# Autodesk Inventor assembly: AssemblyGefreesdBasev2
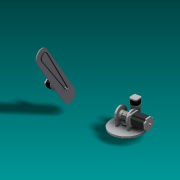
[picture p0: Inventor's stored thumbnail of the model, 180x180]
Saved by Autodesk Inventor 2020.2 (Build 242310000, 310)
## iProperties
Created: 2020-05-18
Part Number: AssemblyGefreesdBasev2
Document SubType Name: Assembly
Designer: Svend
Author: Svend
## Documents named in this file (20)
- C:\Users\Svend\OneDrive\Documents\GitHub\BeerMinder\3D-model\Base (Axis 1)\gefreesd\AssemblyGefreesdBasev2.iam
- C:\Users\Svend\OneDrive\Documents\GitHub\BeerMinder\3D-model\subAssembly\Nema17MetGearbox.iam
- C:\Users\Svend\OneDrive\Documents\GitHub\BeerMinder\3D-model\gearbox\afstandsplaatje.ipt
- C:\Users\Svend\OneDrive\Documents\GitHub\BeerMinder\3D-model\bearings\Ball Bearing 608ZZ.ipt
- C:\Users\Svend\OneDrive\Documents\GitHub\BeerMinder\3D-model\pulleys\GT2 Timing Pulley 20T - 8mm as.ipt
- C:\Users\Svend\OneDrive\Documents\GitHub\BeerMinder\3D-model\pulleys\GT2 Timing Pulley 60T - 8mm as.ipt
- C:\Users\Svend\OneDrive\Documents\GitHub\BeerMinder\3D-model\pulleys\Tandriem20naar60T.ipt
- C:\Users\Svend\OneDrive\Documents\GitHub\BeerMinder\3D-model\Base (Axis 1)\AsBase.ipt
- C:\Users\Svend\OneDrive\Documents\GitHub\BeerMinder\3D-model\subAssembly\Nema23MetGearbox.iam
- C:\Users\Svend\OneDrive\Documents\GitHub\BeerMinder\3D-model\Base (Axis 1)\gefreesd\base bovenkant v2.ipt
- C:\Users\Svend\OneDrive\Documents\GitHub\BeerMinder\3D-model\bearings\51110 Groefkogellager - 70 mm.iam
- C:\Users\Svend\OneDrive\Documents\GitHub\BeerMinder\3D-model\Base (Axis 1)\gefreesd\motorFrame.ipt
- C:\Users\Svend\OneDrive\Documents\GitHub\BeerMinder\3D-model\Base (Axis 1)\gefreesd\base onderkant.ipt
- C:\Users\Svend\OneDrive\Documents\GitHub\BeerMinder\3D-model\Base (Axis 1)\gefreesd\asbevestiging.ipt
- C:\Users\Svend\OneDrive\Documents\GitHub\BeerMinder\3D-model\Base (Axis 1)\gefreesd\gearboxframv2.ipt
- C:\Users\Svend\OneDrive\Documents\Inventor\Content Center Files\R2020\en-US\ISO 7046-1 Z(1)\ISO 7046-1 - M4 x 5 - 4.8 - Z - ISO.ipt
- C:\Users\Svend\OneDrive\Documents\Inventor\Content Center Files\R2020\en-US\ISO 7380-1\ISO 7380-1 - M4 x 12.ipt
- C:\Users\Svend\OneDrive\Documents\Inventor\Content Center Files\R2020\en-US\ISO 7380-1\ISO 7380-1 - M4 x 20.ipt
- C:\Users\Svend\OneDrive\Documents\GitHub\BeerMinder\3D-model\Base (Axis 1)\gefreesd\arm1.ipt
- C:\Users\Svend\OneDrive\Documents\GitHub\BeerMinder\3D-model\pulleys\Tandriem20naar60T-696mm.ipt
## Components (36 placed, 19 different names)
1. base bovenkant v2:1 — Mate:20, Mate:7, Flush:5, Mate:46, Mate:60, Mate:63, Mate:102, Mate:103, Mate:104, Mate:105, Mate:106, Mate:107, Mate:108, Mate:109, Mate:121, Flush:118
2. Nema17MetGearbox:1 [sub-assembly] — Mate:20, Mate:52, Mate:56, Mate:58, Mate:59, Flush:6, Flush:12, Mate:121
3. Ball Bearing 608ZZ:1 — Mate:7, Mate:17, Flush:5, Mate:51
4. GT2 Timing Pulley 20T - 8mm as:1 — Mate:52, Mate:53, Mate:54, Flush:6
5. GT2 Timing Pulley 60T - 8mm as:1 — Mate:14, Mate:40, Mate:51, Mate:55, Flush:15
6. Tandriem20naar60T:1 — Mate:14, Mate:53, Mate:54, Mate:55, Flush:118
7. AsBase:1 — Mate:17, Mate:40, Mate:45, Mate:61, Flush:15, Mate:67
8. Nema23MetGearbox:1 [sub-assembly] — Mate:60, Mate:61, Flush:10, Flush:11, Mate:62, Mate:64, Flush:16, Flush:17, Mate:72, Mate:73
9. 51110 Groefkogellager - 70 mm:1 [sub-assembly] — Mate:45, Mate:46, Mate:71
10. afstandsplaatje:1 — Mate:56, Mate:58, Mate:59, Mate:90, Mate:91, Mate:92, Mate:93
11. motorFrame:1 — Flush:10, Flush:11, Mate:62, Mate:63, Mate:64, Flush:12, Mate:88, Mate:89, Mate:94, Mate:95, Mate:96, Mate:97, Mate:98, Mate:99, Mate:100, Mate:101
12. base onderkant:1 — Mate:67, Mate:68, Mate:69, Mate:70, Mate:71, Mate:110, Mate:111
13. asbevestiging:1 — Mate:68, Mate:69, Mate:70
14. gearboxframv2:1 — Flush:16, Flush:17, Mate:72, Mate:73, Mate:86, Mate:87, Mate:112
15. ISO 7380-1 M4 x 12:1 — Mate:89, Mate:90
16. ISO 7380-1 M4 x 12:2 — Mate:88, Mate:91
17. ISO 7380-1 M4 x 12:3 — Mate:87, Mate:93
18. ISO 7380-1 M4 x 12:4 — Mate:86, Mate:92
19. ISO 7380-1 M4 x 20:1 — Mate:94, Mate:100
20. ISO 7380-1 M4 x 20:2 — Mate:95, Mate:99
21. ISO 7380-1 M4 x 20:4 — Mate:97, Mate:98
22. ISO 7380-1 M4 x 20:3 — Mate:96, Mate:101
23. ISO 7046-1 Z M4 x 5 - 4.8 - Z:5 — Mate:102
24. ISO 7046-1 Z M4 x 5 - 4.8 - Z:6 — Mate:103
25. ISO 7046-1 Z M4 x 5 - 4.8 - Z:7 — Mate:104
26. ISO 7046-1 Z M4 x 5 - 4.8 - Z:8 — Mate:105
27. ISO 7046-1 Z M4 x 5 - 4.8 - Z:9 — Mate:106
28. ISO 7046-1 Z M4 x 5 - 4.8 - Z:10 — Mate:107
29. ISO 7046-1 Z M4 x 5 - 4.8 - Z:11 — Mate:108
30. ISO 7046-1 Z M4 x 5 - 4.8 - Z:12 — Mate:109
31. ISO 7046-1 Z M4 x 5 - 4.8 - Z:13 — Mate:110
32. ISO 7046-1 Z M4 x 5 - 4.8 - Z:14 — Mate:111
33. arm1:1 — Mate:112, Flush:116, Mate:116, Mate:120, Flush:117
34. Nema17MetGearbox:2 [sub-assembly] — Flush:116, Mate:116, Mate:117, Flush:18, Mate:120
35. GT2 Timing Pulley 20T - 8mm as:2 — Mate:117, Flush:18, Mate:118, Mate:119
36. Tandriem20naar60T-696mm:1 — Mate:118, Mate:119, Flush:117
## Relationships (72: Mate 60, Flush 12)
- Mate:20: base bovenkant v2:1 ↔ Nema17MetGearbox:1
- Mate:7: base bovenkant v2:1 ↔ Ball Bearing 608ZZ:1
- Mate:14: GT2 Timing Pulley 60T - 8mm as:1 ↔ Tandriem20naar60T:1
- Mate:17: Ball Bearing 608ZZ:1 ↔ AsBase:1
- Mate:40: GT2 Timing Pulley 60T - 8mm as:1 ↔ AsBase:1
- Flush:5: base bovenkant v2:1 ↔ Ball Bearing 608ZZ:1
- Mate:45: AsBase:1 ↔ 51110 Groefkogellager - 70 mm:1
- Mate:46: base bovenkant v2:1 ↔ 51110 Groefkogellager - 70 mm:1
- Mate:51: Ball Bearing 608ZZ:1 ↔ GT2 Timing Pulley 60T - 8mm as:1
- Mate:52: Nema17MetGearbox:1 ↔ GT2 Timing Pulley 20T - 8mm as:1
- Mate:53 (0.5 mm): GT2 Timing Pulley 20T - 8mm as:1 ↔ Tandriem20naar60T:1
- Mate:54: GT2 Timing Pulley 20T - 8mm as:1 ↔ Tandriem20naar60T:1
- Mate:55 (0.5 mm): GT2 Timing Pulley 60T - 8mm as:1 ↔ Tandriem20naar60T:1
- Mate:56: Nema17MetGearbox:1 ↔ afstandsplaatje:1
- Mate:58: Nema17MetGearbox:1 ↔ afstandsplaatje:1
- Mate:59: Nema17MetGearbox:1 ↔ afstandsplaatje:1
- Flush:6: Nema17MetGearbox:1 ↔ GT2 Timing Pulley 20T - 8mm as:1
- Mate:60 (20 mm): base bovenkant v2:1 ↔ Nema23MetGearbox:1
- Mate:61 (-29.76 mm): AsBase:1 ↔ Nema23MetGearbox:1
- Flush:10: Nema23MetGearbox:1 ↔ motorFrame:1
- Flush:11: Nema23MetGearbox:1 ↔ motorFrame:1
- Mate:62: Nema23MetGearbox:1 ↔ motorFrame:1
- Mate:63: base bovenkant v2:1 ↔ motorFrame:1
- Mate:64: Nema23MetGearbox:1 ↔ motorFrame:1
- Flush:12 (-26.25 mm): Nema17MetGearbox:1 ↔ motorFrame:1
- Flush:15: GT2 Timing Pulley 60T - 8mm as:1 ↔ AsBase:1
- Mate:67: AsBase:1 ↔ base onderkant:1
- Mate:68: base onderkant:1 ↔ asbevestiging:1
- Mate:69: base onderkant:1 ↔ asbevestiging:1
- Mate:70: base onderkant:1 ↔ asbevestiging:1
- Flush:16: Nema23MetGearbox:1 ↔ gearboxframv2:1
- Flush:17: Nema23MetGearbox:1 ↔ gearboxframv2:1
- Mate:71: 51110 Groefkogellager - 70 mm:1 ↔ base onderkant:1
- Mate:72: Nema23MetGearbox:1 ↔ gearboxframv2:1
- Mate:73: Nema23MetGearbox:1 ↔ gearboxframv2:1
- Mate:86: gearboxframv2:1 ↔ ISO 7380-1 M4 x 12:4
- Mate:87: gearboxframv2:1 ↔ ISO 7380-1 M4 x 12:3
- Mate:88: motorFrame:1 ↔ ISO 7380-1 M4 x 12:2
- Mate:89: motorFrame:1 ↔ ISO 7380-1 M4 x 12:1
- Mate:90: afstandsplaatje:1 ↔ ISO 7380-1 M4 x 12:1
- Mate:91: afstandsplaatje:1 ↔ ISO 7380-1 M4 x 12:2
- Mate:92: afstandsplaatje:1 ↔ ISO 7380-1 M4 x 12:4
- Mate:93: afstandsplaatje:1 ↔ ISO 7380-1 M4 x 12:3
- Mate:94: motorFrame:1 ↔ ISO 7380-1 M4 x 20:1
- Mate:95: motorFrame:1 ↔ ISO 7380-1 M4 x 20:2
- Mate:96: motorFrame:1 ↔ ISO 7380-1 M4 x 20:3
- Mate:97: motorFrame:1 ↔ ISO 7380-1 M4 x 20:4
- Mate:98: motorFrame:1 ↔ ISO 7380-1 M4 x 20:4
- Mate:99: motorFrame:1 ↔ ISO 7380-1 M4 x 20:2
- Mate:100: motorFrame:1 ↔ ISO 7380-1 M4 x 20:1
- Mate:101: motorFrame:1 ↔ ISO 7380-1 M4 x 20:3
- Mate:102: base bovenkant v2:1 ↔ ISO 7046-1 Z M4 x 5 - 4.8 - Z:5
- Mate:103: base bovenkant v2:1 ↔ ISO 7046-1 Z M4 x 5 - 4.8 - Z:6
- Mate:104: base bovenkant v2:1 ↔ ISO 7046-1 Z M4 x 5 - 4.8 - Z:7
- Mate:105: base bovenkant v2:1 ↔ ISO 7046-1 Z M4 x 5 - 4.8 - Z:8
- Mate:106: base bovenkant v2:1 ↔ ISO 7046-1 Z M4 x 5 - 4.8 - Z:9
- Mate:107: base bovenkant v2:1 ↔ ISO 7046-1 Z M4 x 5 - 4.8 - Z:10
- Mate:108: base bovenkant v2:1 ↔ ISO 7046-1 Z M4 x 5 - 4.8 - Z:11
- Mate:109: base bovenkant v2:1 ↔ ISO 7046-1 Z M4 x 5 - 4.8 - Z:12
- Mate:110: base onderkant:1 ↔ ISO 7046-1 Z M4 x 5 - 4.8 - Z:13
- Mate:111: base onderkant:1 ↔ ISO 7046-1 Z M4 x 5 - 4.8 - Z:14
- Mate:112: gearboxframv2:1 ↔ arm1:1
- Flush:116: arm1:1 ↔ Nema17MetGearbox:2
- Mate:116: arm1:1 ↔ Nema17MetGearbox:2
- Mate:117: Nema17MetGearbox:2 ↔ GT2 Timing Pulley 20T - 8mm as:2
- Flush:18 (-2 mm): Nema17MetGearbox:2 ↔ GT2 Timing Pulley 20T - 8mm as:2
- Mate:118: GT2 Timing Pulley 20T - 8mm as:2 ↔ Tandriem20naar60T-696mm:1
- Mate:119 (0.5 mm): GT2 Timing Pulley 20T - 8mm as:2 ↔ Tandriem20naar60T-696mm:1
- Mate:120 (60 mm): arm1:1 ↔ Nema17MetGearbox:2
- Flush:117: arm1:1 ↔ Tandriem20naar60T-696mm:1
- Mate:121: base bovenkant v2:1 ↔ Nema17MetGearbox:1
- Flush:118: base bovenkant v2:1 ↔ Tandriem20naar60T:1
